# Autodesk Inventor assembly: manipulator assembly
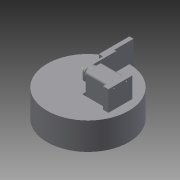
[picture p0: Inventor's stored thumbnail of the model, 180x180]
Saved by Autodesk Inventor 2015 (Build 190159000, 159)
## iProperties
Created: 2014-10-22
Part Number: manipulator assembly
Document SubType Name: Assembly
Designer: ericd_000
Author: ericd_000
## Documents named in this file (4)
- C:\Users\ericd_000\Dropbox\GitHub\initial_cad\eric_cad\manipulator assembly.iam
- C:\Users\ericd_000\Dropbox\GitHub\initial_cad\eric_cad\manipulator base.ipt
- C:\Users\ericd_000\Dropbox\GitHub\initial_cad\eric_cad\herkulex assembled.iam
- C:\Users\ericd_000\Dropbox\GitHub\initial_cad\eric_cad\first_man_link.ipt
## Components (3 placed, 3 different names)
1. manipulator base:1 — Rotational:1, Rotational:2
2. herkulex assembled:1 [sub-assembly] — Rotational:1, Rotational:2, Mate:1, Rotational:3
3. first_man_link:1 — Mate:1, Rotational:3
## Relationships (4: RevoluteJoint 3, Mate 1)
- Rotational:1 [RevoluteJoint]: manipulator base:1 ↔ herkulex assembled:1
- Rotational:2 [RevoluteJoint]: manipulator base:1 ↔ herkulex assembled:1
- Mate:1: herkulex assembled:1 ↔ first_man_link:1
- Rotational:3 [RevoluteJoint]: herkulex assembled:1 ↔ first_man_link:1
